# Autodesk Inventor assembly: joint assembly
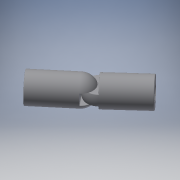
[picture p0: Inventor's stored thumbnail of the model, 180x180]
Saved by Autodesk Inventor 2018 (Build 220112000, 112)
## iProperties
Created: 2018-04-05
Part Number: joint assembly
Document SubType Name: Assembly
Designer: 232963
Author: 232963
## Documents named in this file (3)
- P:\IED\SchoolCAD\Design Challenge\joint assembly.iam
- P:\IED\SchoolCAD\Design Challenge\joint 1.ipt
- P:\IED\SchoolCAD\Design Challenge\joint 2.ipt
## Components (2 placed, 2 different names)
1. joint 1:1 — Insert:1
2. joint 2:1 — Insert:1
## Relationships (1: Insert 1)
- Insert:1: joint 1:1 ↔ joint 2:1
